# Autodesk Inventor assembly: 装配体2_MIR1
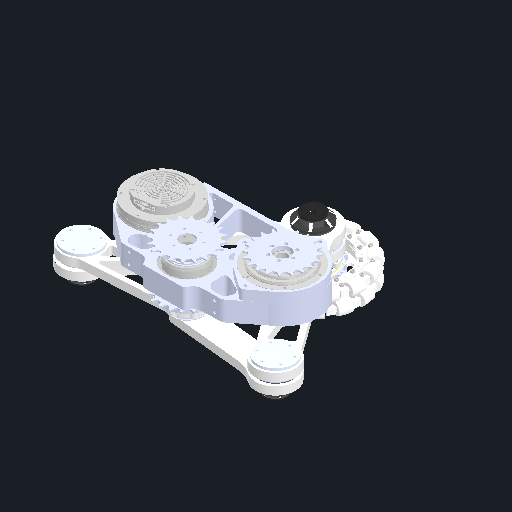
[picture p0: Inventor's stored thumbnail of the model, 512x512]
Saved by Autodesk Inventor 2025 (Build 290162000, 162)
## iProperties
Created: 2025-03-28
Part Number: 装配体2_MIR1
Document SubType Name: Assembly
Designer: XH
Author: XH
Sending System: SolidWorks 2018
Last Author: Standard
Last Saved: 2025-04-01
代号代码: Assembly.Extension.CustomPropertyManager("").Set("代号",Left(Assembly.GetTitle,InStr(Assembly.GetTitle," ")-1))
名称代码: Assembly.Extension.CustomPropertyManager("").Set("名称",Right(Assembly.GetTitle,Len(Assembly.GetTitle)-InStr(Assembly.GetTitle," ")))
日期: 1800-01-01
名称: 装配体2
Weight: 12.94
版本号: a.1
图样标记S: S
基本计量单位（必填）: 个
## Documents named in this file (23)
- C:\1A_Engineering_files\RCInventor\铝件版本\装配体2_MIR1.iam
- C:\1A_Engineering_files\RCInventor\铝件版本\零件6_MIR1.ipt
- C:\1A_Engineering_files\RCInventor\铝件版本\BAR6806_MIR1.ipt
- C:\1A_Engineering_files\RCInventor\铝件版本\零件1_MIR1.ipt
- C:\1A_Engineering_files\RCInventor\铝件版本\61810_MIR1.ipt
- C:\1A_Engineering_files\RCInventor\铝件版本\2_MIR1.ipt
- C:\1A_Engineering_files\RCInventor\铝件版本\零件4_MIR1.ipt
- C:\1A_Engineering_files\RCInventor\铝件版本\碗组\标件_碗组总成_MIR1.iam
- C:\1A_Engineering_files\RCInventor\铝件版本\碗组\机加工_碗组连接1_MIR1.ipt
- C:\1A_Engineering_files\RCInventor\铝件版本\碗组\碗组_培林总成_MIR1.ipt
- C:\1A_Engineering_files\RCInventor\铝件版本\碗组\碗组_下底_MIR1.ipt
- C:\1A_Engineering_files\RCInventor\铝件版本\碗组\板材_垫块_MIR1.ipt
- C:\1A_Engineering_files\RCInventor\铝件版本\机加件-髋关节复合固定件_MIR1.ipt
- C:\1A_Engineering_files\RCInventor\铝件版本\dm8009-20240822_MIR1.iam
- C:\1A_Engineering_files\RCInventor\铝件版本\31231_MIR1.ipt
- C:\1A_Engineering_files\RCInventor\铝件版本\链条\机加件-右关节链轮-20H04A_MIR1.ipt
- C:\1A_Engineering_files\RCInventor\铝件版本\链条\机加件-大腿驱动链轮-20H04A_MIR1.ipt
- C:\1A_Engineering_files\RCInventor\铝件版本\链条\机加件-右关节链轮-20H04A2_MIR1.ipt
- C:\1A_Engineering_files\RCInventor\铝件版本\链条\机加件-大腿驱动链轮-20H04A2_MIR1.ipt
- C:\1A_Engineering_files\RCInventor\铝件版本\链条\标准件-推力轴承52-35-h4_MIR1.ipt
- C:\1A_Engineering_files\RCInventor\铝件版本\链条\碳纤维(cnc)-关节电机端子延展_MIR1.ipt
- C:\1A_Engineering_files\RCInventor\铝件版本\轮系\客户模型 M3508减速箱 减比268：17.iam
- C:\1A_Engineering_files\RCInventor\铝件版本\机加工_轮轴加工.ipt
## Components (34 placed, 22 different names)
1. 零件6_MIR1:1 — 配合:53, 配合:47, 配合:45, 配合:44, 配合:101, 配合:88, 配合:8, 配合:103, 配合:100, 配合:79, 配合:86, 配合:106
2. BAR6806_MIR1:1 — 配合:53, 配合:47, 配合:51
3. 零件1_MIR1:1 — 配合:51, 配合:45, 配合:59, 配合:46, 配合:49, 配合:48, 配合:56, 配合:81
4. 61810_MIR1:1 — 配合:44, 配合:58
5. 61810_MIR1:2 — 配合:59, 配合:46, 配合:73
6. 2_MIR1:1 — 配合:49, 配合:48, 配合:36, 配合:35, 配合:34, 配合:80, 配合:87
7. 零件4_MIR1:1 — 配合:101, 配合:88, 配合:8, 配合:63, 配合:5, 配合:9, 配合:64
8. 标件_碗组总成_MIR1:1 [sub-assembly] — 配合:63, 配合:5, 配合:10, 配合:62
9. 机加工_碗组连接1_MIR1:1 — 配合:10, 配合:9, 配合:17, 配合:68, 配合:65
10. 碗组_培林总成_MIR1:1 — 配合:64, 配合:62, 配合:13, 配合:12
11. 碗组_下底_MIR1:1 — 配合:13, 配合:12
12. 板材_垫块_MIR1:1 — 配合:17, 配合:66
13. 标件_碗组总成_MIR1:2 [sub-assembly] — 配合:82, 配合:37, 配合:83, 配合:95, 配合:94
14. 机加工_碗组连接1_MIR1:2 — 配合:82, 配合:37, 配合:36, 配合:35, 配合:31, 配合:30
15. 碗组_培林总成_MIR1:2 — 配合:83, 配合:31, 配合:29, 配合:28
16. 碗组_下底_MIR1:2 — 配合:29, 配合:28
17. 板材_垫块_MIR1:2 — 配合:34, 配合:30
18. 机加件-髋关节复合固定件_MIR1:1 — 配合:73, 配合:58, 配合:56, 配合:90, 配合:55, 配合:54
19. dm8009-20240822_MIR1:1 [sub-assembly] — 配合:90, 配合:99, 配合:98, 配合:107
20. dm8009-20240822_MIR1:2 [sub-assembly] — 配合:55, 配合:54, 配合:102, 配合:71
21. 31231_MIR1:1 — 配合:68, 配合:66, 配合:65, 配合:96, 配合:72
22. 机加件-右关节链轮-20H04A_MIR1:1 — 配合:102, 配合:71, 表面齐平:5
23. 机加件-大腿驱动链轮-20H04A_MIR1:1 — 表面齐平:5, 配合:81, 配合:80, 表面齐平:3, 配合:78
24. 机加件-右关节链轮-20H04A2_MIR1:1 — 配合:99, 配合:98, 表面齐平:4
25. 机加件-大腿驱动链轮-20H04A2_MIR1:1 — 配合:103, 配合:100, 表面齐平:4
26. BAR6806_MIR1:2 — 配合:79, 表面齐平:3, 配合:78
27. 标准件-推力轴承52-35-h4_MIR1:1 — 配合:87, 配合:86
28. 31231_MIR1:2 — 配合:96, 配合:95, 配合:94, 配合:66, 配合:75, 配合:76
29. 标准件-推力轴承52-35-h4_MIR1:3 — 配合:106
30. 碳纤维(cnc)-关节电机端子延展_MIR1:1 — 配合:107
31. 客户模型 M3508减速箱 减比268：17:1 [sub-assembly] — 配合:66, 配合:73, 配合:74, 配合:76
32. 标件_碗组总成_MIR1:3 [sub-assembly]
33. 碗组_培林总成_MIR1:3 — 配合:72
34. 机加工_轮轴加工:1 — 配合:73, 配合:74, 配合:75
## Relationships (67: Mate 64, Flush 3)
- 配合:53 [Mate]: 零件6_MIR1:1 ↔ BAR6806_MIR1:1
- 配合:47 [Mate]: 零件6_MIR1:1 ↔ BAR6806_MIR1:1
- 配合:51 [Mate]: BAR6806_MIR1:1 ↔ 零件1_MIR1:1
- 配合:45 [Mate]: 零件6_MIR1:1 ↔ 零件1_MIR1:1
- 配合:44 [Mate]: 零件6_MIR1:1 ↔ 61810_MIR1:1
- 配合:59 [Mate]: 零件1_MIR1:1 ↔ 61810_MIR1:2
- 配合:46 [Mate]: 零件1_MIR1:1 ↔ 61810_MIR1:2
- 配合:49 [Mate]: 零件1_MIR1:1 ↔ 2_MIR1:1
- 配合:48 [Mate]: 零件1_MIR1:1 ↔ 2_MIR1:1
- 配合:101 [Mate]: 零件6_MIR1:1 ↔ 零件4_MIR1:1
- 配合:88 [Mate]: 零件6_MIR1:1 ↔ 零件4_MIR1:1
- 配合:8 [Mate]: 零件6_MIR1:1 ↔ 零件4_MIR1:1
- 配合:63 [Mate]: 零件4_MIR1:1 ↔ 标件_碗组总成_MIR1:1
- 配合:5 [Mate]: 零件4_MIR1:1 ↔ 标件_碗组总成_MIR1:1
- 配合:10 [Mate]: 标件_碗组总成_MIR1:1 ↔ 机加工_碗组连接1_MIR1:1
- 配合:9 [Mate]: 零件4_MIR1:1 ↔ 机加工_碗组连接1_MIR1:1
- 配合:64 [Mate]: 零件4_MIR1:1 ↔ 碗组_培林总成_MIR1:1
- 配合:62 [Mate]: 标件_碗组总成_MIR1:1 ↔ 碗组_培林总成_MIR1:1
- 配合:13 [Mate]: 碗组_培林总成_MIR1:1 ↔ 碗组_下底_MIR1:1
- 配合:12 [Mate]: 碗组_培林总成_MIR1:1 ↔ 碗组_下底_MIR1:1
- 配合:17 [Mate]: 机加工_碗组连接1_MIR1:1 ↔ 板材_垫块_MIR1:1
- 配合:82 [Mate]: 标件_碗组总成_MIR1:2 ↔ 机加工_碗组连接1_MIR1:2
- 配合:37 [Mate]: 标件_碗组总成_MIR1:2 ↔ 机加工_碗组连接1_MIR1:2
- 配合:36 [Mate]: 2_MIR1:1 ↔ 机加工_碗组连接1_MIR1:2
- 配合:35 [Mate]: 2_MIR1:1 ↔ 机加工_碗组连接1_MIR1:2
- 配合:83 [Mate]: 标件_碗组总成_MIR1:2 ↔ 碗组_培林总成_MIR1:2
- 配合:31 [Mate]: 机加工_碗组连接1_MIR1:2 ↔ 碗组_培林总成_MIR1:2
- 配合:29 [Mate]: 碗组_培林总成_MIR1:2 ↔ 碗组_下底_MIR1:2
- 配合:28 [Mate]: 碗组_培林总成_MIR1:2 ↔ 碗组_下底_MIR1:2
- 配合:34 [Mate]: 2_MIR1:1 ↔ 板材_垫块_MIR1:2
- 配合:30 [Mate]: 机加工_碗组连接1_MIR1:2 ↔ 板材_垫块_MIR1:2
- 配合:73 [Mate]: 61810_MIR1:2 ↔ 机加件-髋关节复合固定件_MIR1:1
- 配合:58 [Mate]: 61810_MIR1:1 ↔ 机加件-髋关节复合固定件_MIR1:1
- 配合:56 [Mate]: 零件1_MIR1:1 ↔ 机加件-髋关节复合固定件_MIR1:1
- 配合:90 [Mate]: 机加件-髋关节复合固定件_MIR1:1 ↔ dm8009-20240822_MIR1:1
- 配合:55 [Mate]: 机加件-髋关节复合固定件_MIR1:1 ↔ dm8009-20240822_MIR1:2
- 配合:54 [Mate]: 机加件-髋关节复合固定件_MIR1:1 ↔ dm8009-20240822_MIR1:2
- 配合:68 [Mate]: 机加工_碗组连接1_MIR1:1 ↔ 31231_MIR1:1
- 配合:66 [Mate]: 板材_垫块_MIR1:1 ↔ 31231_MIR1:1
- 配合:65 [Mate]: 机加工_碗组连接1_MIR1:1 ↔ 31231_MIR1:1
- 配合:102 [Mate]: dm8009-20240822_MIR1:2 ↔ 机加件-右关节链轮-20H04A_MIR1:1
- 配合:71 [Mate]: dm8009-20240822_MIR1:2 ↔ 机加件-右关节链轮-20H04A_MIR1:1
- 表面齐平:5 [Flush]: 机加件-右关节链轮-20H04A_MIR1:1 ↔ 机加件-大腿驱动链轮-20H04A_MIR1:1
- 配合:81 [Mate]: 零件1_MIR1:1 ↔ 机加件-大腿驱动链轮-20H04A_MIR1:1
- 配合:80 [Mate]: 2_MIR1:1 ↔ 机加件-大腿驱动链轮-20H04A_MIR1:1
- 配合:99 [Mate]: dm8009-20240822_MIR1:1 ↔ 机加件-右关节链轮-20H04A2_MIR1:1
- 配合:98 [Mate]: dm8009-20240822_MIR1:1 ↔ 机加件-右关节链轮-20H04A2_MIR1:1
- 配合:103 [Mate]: 零件6_MIR1:1 ↔ 机加件-大腿驱动链轮-20H04A2_MIR1:1
- 配合:100 [Mate]: 零件6_MIR1:1 ↔ 机加件-大腿驱动链轮-20H04A2_MIR1:1
- 表面齐平:4 [Flush]: 机加件-右关节链轮-20H04A2_MIR1:1 ↔ 机加件-大腿驱动链轮-20H04A2_MIR1:1
- 配合:79 [Mate]: 零件6_MIR1:1 ↔ BAR6806_MIR1:2
- 表面齐平:3 [Flush]: 机加件-大腿驱动链轮-20H04A_MIR1:1 ↔ BAR6806_MIR1:2
- 配合:78 [Mate]: 机加件-大腿驱动链轮-20H04A_MIR1:1 ↔ BAR6806_MIR1:2
- 配合:87 [Mate]: 2_MIR1:1 ↔ 标准件-推力轴承52-35-h4_MIR1:1
- 配合:86 [Mate]: 零件6_MIR1:1 ↔ 标准件-推力轴承52-35-h4_MIR1:1
- 配合:96 [Mate]: 31231_MIR1:1 ↔ 31231_MIR1:2
- 配合:95 [Mate]: 标件_碗组总成_MIR1:2 ↔ 31231_MIR1:2
- 配合:94 [Mate]: 标件_碗组总成_MIR1:2 ↔ 31231_MIR1:2
- 配合:106 [Mate]: 零件6_MIR1:1 ↔ 标准件-推力轴承52-35-h4_MIR1:3
- 配合:107 [Mate]: dm8009-20240822_MIR1:1 ↔ 碳纤维(cnc)-关节电机端子延展_MIR1:1
- 配合:66 [Mate]: 31231_MIR1:2 ↔ 客户模型 M3508减速箱 减比268：17:1
- [Mate]: 标件_碗组总成_MIR1:3 ↔ 碗组_培林总成_MIR1:3
- 配合:72 [Mate]: 31231_MIR1:1 ↔ 碗组_培林总成_MIR1:3
- 配合:73 [Mate]: 客户模型 M3508减速箱 减比268：17:1 ↔ 机加工_轮轴加工:1
- 配合:74 [Mate]: 客户模型 M3508减速箱 减比268：17:1 ↔ 机加工_轮轴加工:1
- 配合:75 [Mate]: 31231_MIR1:2 ↔ 机加工_轮轴加工:1
- 配合:76 [Mate] (10 mm): 31231_MIR1:2 ↔ 客户模型 M3508减速箱 减比268：17:1
## Named parameters: d73_d17 = 0 mm
